# Autodesk Inventor assembly: assembly
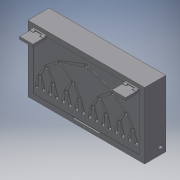
[picture p0: Inventor's stored thumbnail of the model, 180x180]
Saved by Autodesk Inventor 2018.2 (Build 222227000, 227)
## iProperties
Created: 2018-03-24
Part Number: assembly
Document SubType Name: Assembly
Designer: wharr
Author: wharr
## Documents named in this file (4)
- C:\MEGA\NCSSM\CS434 Data Structures I\neopixel-bst\parts\assembly.iam
- C:\MEGA\NCSSM\CS434 Data Structures I\neopixel-bst\parts\housing.ipt
- C:\MEGA\NCSSM\CS434 Data Structures I\neopixel-bst\parts\hinge.ipt
- C:\MEGA\NCSSM\CS434 Data Structures I\neopixel-bst\parts\front plate.ipt
## Components (4 placed, 3 different names)
1. housing:1 — Mate:1, Mate:2, Mate:3, Mate:4, Mate:5, Mate:6, Mate:7, Mate:8, Mate:9
2. hinge:1 — Mate:1, Mate:2, Mate:3
3. hinge:2 — Mate:4, Mate:5, Mate:6
4. front plate:1 — Mate:7, Mate:8, Mate:9
## Relationships (9: Mate 9)
- Mate:1: housing:1 ↔ hinge:1
- Mate:2: housing:1 ↔ hinge:1
- Mate:3: housing:1 ↔ hinge:1
- Mate:4: housing:1 ↔ hinge:2
- Mate:5: housing:1 ↔ hinge:2
- Mate:6: housing:1 ↔ hinge:2
- Mate:7: housing:1 ↔ front plate:1
- Mate:8: housing:1 ↔ front plate:1
- Mate:9: housing:1 ↔ front plate:1
